# Autodesk Inventor assembly: Arm
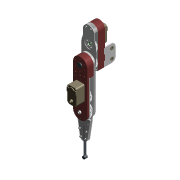
[picture p0: Inventor's stored thumbnail of the model, 180x180]
Saved by Autodesk Inventor 2013 (Build 170138000, 138)
## iProperties
Created: 2013-02-07
Part Number: Arm
Document SubType Name: Assembly
Designer: JohnHenry
Mass: 271.096 g
Surface Area: 817.136 cm^2
Volume: 121.712 cm^3
Density: 2.22735 g/cm^3
Author: JohnHenry
## Documents named in this file (23)
- C:\Users\victor\Desktop\Documents\Inventor\walkPivot\Arm.iam
- C:\Users\victor\Desktop\Documents\Inventor\walkPivot\JointC3_2nd.ipt
- C:\Users\victor\Desktop\Documents\Inventor\walkPivot\JointC3'_2nd.ipt
- C:\Users\victor\Desktop\Documents\Inventor\walkPivot\ベアリング(仮).ipt
- C:\Users\victor\Desktop\Documents\Inventor\walkPivot\RS30x_BottomShaft.ipt
- C:\Users\victor\Desktop\Documents\Inventor\walkPivot\RS30x_ServoHorn.ipt
- C:\Users\victor\Desktop\Documents\Inventor\walkPivot\S75B 40B+0306\デザイン アクセラレータ\平歯車11.ipt
- C:\Users\victor\Desktop\Documents\Inventor\walkPivot\JointC3'cover_2nd.ipt
- C:\Users\victor\Desktop\Documents\Inventor\walkPivot\JointC2_2nd.ipt
- C:\Users\victor\Desktop\Documents\Inventor\walkPivot\S75B 40B+0306\デザイン アクセラレータ\平歯車11_.ipt
- C:\Users\victor\Desktop\Documents\Inventor\walkPivot\JointC3'B_2nd.ipt
- C:\Users\victor\Desktop\Documents\Inventor\walkPivot\JointD0_2nd.ipt
- C:\Users\victor\Desktop\Documents\Inventor\walkPivot\S75B 40B+0306\デザイン アクセラレータ\平歯車11__.ipt
- C:\Users\victor\Desktop\Documents\Inventor\walkPivot\JointD2_2nd.ipt
- C:\Users\victor\Desktop\Documents\Inventor\walkPivot\JointC2cover_2nd.ipt
- C:\Users\victor\Desktop\Documents\Inventor\walkPivot\M2_5mm.ipt
- C:\Users\victor\Desktop\Documents\Inventor\walkPivot\M3_10.ipt
- C:\Users\victor\Desktop\Documents\Inventor\walkPivot\80F-0605.ipt
- C:\Users\victor\Desktop\Documents\Inventor\walkPivot\M1.6_5mm.ipt
- C:\Users\victor\Desktop\Documents\Inventor\walkPivot\shaft6-47.8.ipt
- C:\Users\victor\Desktop\Documents\Inventor\walkPivot\shaft6-19.ipt
- C:\Users\victor\Desktop\Documents\Inventor\walkPivot\JointD0cover_2nd.ipt
- C:\Users\victor\Desktop\Documents\Inventor\walkPivot\JointC3'cover2_2nd.ipt
## Components (81 placed, 20 different names)
1. JointC3_2nd:1 — 挿入:1, 挿入:2, 挿入:3, 挿入:4, 挿入:5, 挿入:6, 挿入:70, 挿入:71, 挿入:72, 挿入:73
2. JointC3'_2nd:1 — 挿入:5, 挿入:6, メイト:2, 角度:1, 挿入:9, 挿入:10, メイト:3, メイト:6, フラッシュ:3, 角度:5, 挿入:60
3. ベアリング(仮):1 — 挿入:3
4. ベアリング(仮):2 — 挿入:2
5. ベアリング(仮):3 — 挿入:4
6. ベアリング(仮):4 — 挿入:1
7. RS30x_BottomShaft:1 — メイト:2, メイト:6, フラッシュ:3, 挿入:13
8. RS30x_ServoHorn:1 — 角度:1, 角度:2, 挿入:8, 挿入:13
9. 平歯車1:1 — 角度:2, 挿入:8, フラッシュ:2, 挿入:66, 挿入:67, 挿入:68, 挿入:69
10. JointC3'cover_2nd:1 — 挿入:9, 挿入:10, 挿入:38, 挿入:39, 挿入:40, 挿入:41, 挿入:53, 挿入:54, 挿入:61, 挿入:86, 挿入:87, 挿入:90, 挿入:91
11. JointC2_2nd:1 — 挿入:11, 挿入:12, メイト:4, メイト:5, フラッシュ:4, 挿入:16, 挿入:17, メイト:7, 角度:5, 角度:6, 挿入:24, 挿入:25, 挿入:74, 挿入:96
12. 平歯車1:2 — メイト:3, フラッシュ:2, 挿入:11, 挿入:12, 挿入:44, 挿入:45, 挿入:46, 挿入:47, 挿入:48, 挿入:49
13. RS30x_BottomShaft:2 — メイト:4, メイト:5, フラッシュ:4, 挿入:14
14. RS30x_ServoHorn:2 — 挿入:14, 角度:4, 挿入:20
15. 平歯車1:3 — 角度:4, フラッシュ:5, 挿入:20, 挿入:62, 挿入:63, 挿入:64, 挿入:65
16. JointC3'B_2nd:1 — 挿入:16, 挿入:17, 挿入:55, 挿入:56, 挿入:57
17. JointD0_2nd:1 — 挿入:18, 挿入:19, フラッシュ:6, メイト:8, メイト:9, 挿入:23, 挿入:26, 挿入:27, 挿入:28, 挿入:29, 挿入:76, 挿入:77, 挿入:78, 挿入:79, 挿入:92
18. 平歯車1:4 — メイト:7, フラッシュ:5, 挿入:18, 挿入:19, 挿入:95
19. JointD2_2nd:1 — フラッシュ:6, メイト:8, メイト:9, 角度:6
20. JointC2cover_2nd:1 — 挿入:24, 挿入:25, 挿入:30, 挿入:31, 挿入:32, 挿入:33, 挿入:34, 挿入:50, 挿入:51, 挿入:52, 挿入:88, 挿入:89
21. M2_5mm:1 — 挿入:31
22. M2_5mm:2 — 挿入:28
23. M2_5mm:3 — 挿入:29
24. M2_5mm:4 — 挿入:32
25. M2_5mm:5 — 挿入:41
26. M2_5mm:6 — 挿入:40
27. M2_5mm:7 — 挿入:33
28. M2_5mm:8 — 挿入:52
29. M2_5mm:9 — 挿入:34
30. M2_5mm:10 — 挿入:30
31. M2_5mm:11 — 挿入:26
32. M2_5mm:12 — 挿入:27
33. M2_5mm:13 — 挿入:50
34. M2_5mm:15 — 挿入:38
35. M2_5mm:16 — 挿入:23
36. M2_5mm:17 — 挿入:39
37. M2_5mm:18 — 挿入:51
38. M2_5mm:20 — 挿入:49
39. M2_5mm:21 — 挿入:48
40. M2_5mm:25 — 挿入:45
41. M2_5mm:26 — 挿入:44
42. M2_5mm:27 — 挿入:47
43. M2_5mm:28 — 挿入:46
44. M2_5mm:29 — 挿入:54
45. M2_5mm:30 — 挿入:53
46. M3_10:1 — 挿入:55
47. M3_10:2 — 挿入:56
48. M3_10:3 — 挿入:57
49. 80F-0605:1 — 挿入:95
50. 80F-0605:3 — 挿入:61
51. 80F-0605:4 — 挿入:60
52. M1.6_5mm:1 — 挿入:62
53. M1.6_5mm:2 — 挿入:64
54. M1.6_5mm:3 — 挿入:65
55. M1.6_5mm:4 — 挿入:63
56. M1.6_5mm:5 — 挿入:67
57. M1.6_5mm:6 — 挿入:66
58. M1.6_5mm:7 — 挿入:68
59. M1.6_5mm:8 — 挿入:69
60. M3_10:4 — 挿入:71
61. M3_10:5 — 挿入:70
62. M3_10:6 — 挿入:73
63. M3_10:7 — 挿入:72
64. shaft6-47.8:1 — 挿入:74
65. shaft6-19:1 — 挿入:96, 挿入:97, 挿入:98
66. JointD0cover_2nd:1 — 挿入:78, 挿入:79, 挿入:81, 挿入:82, 挿入:84, 挿入:85
67. JointD0cover_2nd:2 — 挿入:76, 挿入:77
68. M2_5mm:31 — 挿入:85
69. M2_5mm:32 — 挿入:84
70. M2_5mm:35 — 挿入:81
71. M2_5mm:36 — 挿入:82
72. JointC3'cover2_2nd:1 — 挿入:86, 挿入:87, 挿入:93, 挿入:94
73. M2_5mm:37 — 挿入:89
74. M2_5mm:38 — 挿入:88
75. M2_5mm:39 — 挿入:90
76. M2_5mm:40 — 挿入:91
77. M2_5mm:41 — 挿入:92
78. M2_5mm:42 — 挿入:94
79. M2_5mm:43 — 挿入:93
80. M3_10:8 — 挿入:97
81. M3_10:9 — 挿入:98
## Relationships (102: Insert 84, Mate 8, Angle 5, Flush 5)
- 挿入:1 [Insert]: JointC3_2nd:1 ↔ ベアリング(仮):4
- 挿入:2 [Insert]: JointC3_2nd:1 ↔ ベアリング(仮):2
- 挿入:3 [Insert]: JointC3_2nd:1 ↔ ベアリング(仮):1
- 挿入:4 [Insert]: JointC3_2nd:1 ↔ ベアリング(仮):3
- 挿入:5 [Insert]: JointC3_2nd:1 ↔ JointC3'_2nd:1
- 挿入:6 [Insert]: JointC3_2nd:1 ↔ JointC3'_2nd:1
- メイト:2 [Mate] (0.05 mm): JointC3'_2nd:1 ↔ RS30x_BottomShaft:1
- 角度:1 [Angle] (0 deg): JointC3'_2nd:1 ↔ RS30x_ServoHorn:1
- 角度:2 [Angle] (0 deg): RS30x_ServoHorn:1 ↔ 平歯車1:1
- 挿入:8 [Insert]: RS30x_ServoHorn:1 ↔ 平歯車1:1
- 挿入:9 [Insert]: JointC3'_2nd:1 ↔ JointC3'cover_2nd:1
- 挿入:10 [Insert]: JointC3'_2nd:1 ↔ JointC3'cover_2nd:1
- メイト:3 [Mate]: JointC3'_2nd:1 ↔ 平歯車1:2
- フラッシュ:2 [Flush]: 平歯車1:1 ↔ 平歯車1:2
- 挿入:11 [Insert]: JointC2_2nd:1 ↔ 平歯車1:2
- 挿入:12 [Insert]: JointC2_2nd:1 ↔ 平歯車1:2
- メイト:4 [Mate] (0.05 mm): JointC2_2nd:1 ↔ RS30x_BottomShaft:2
- メイト:5 [Mate] (0.05 mm): JointC2_2nd:1 ↔ RS30x_BottomShaft:2
- メイト:6 [Mate] (0.05 mm): JointC3'_2nd:1 ↔ RS30x_BottomShaft:1
- フラッシュ:3 [Flush]: JointC3'_2nd:1 ↔ RS30x_BottomShaft:1
- 挿入:13 [Insert]: RS30x_BottomShaft:1 ↔ RS30x_ServoHorn:1
- フラッシュ:4 [Flush]: JointC2_2nd:1 ↔ RS30x_BottomShaft:2
- 挿入:14 [Insert]: RS30x_BottomShaft:2 ↔ RS30x_ServoHorn:2
- 角度:4 [Angle] (0 deg): RS30x_ServoHorn:2 ↔ 平歯車1:3
- 挿入:16 [Insert]: JointC2_2nd:1 ↔ JointC3'B_2nd:1
- 挿入:17 [Insert]: JointC2_2nd:1 ↔ JointC3'B_2nd:1
- メイト:7 [Mate]: JointC2_2nd:1 ↔ 平歯車1:4
- フラッシュ:5 [Flush]: 平歯車1:3 ↔ 平歯車1:4
- 挿入:18 [Insert]: JointD0_2nd:1 ↔ 平歯車1:4
- 挿入:19 [Insert]: JointD0_2nd:1 ↔ 平歯車1:4
- 角度:5 [Angle] (0 deg): JointC3'_2nd:1 ↔ JointC2_2nd:1
- フラッシュ:6 [Flush]: JointD0_2nd:1 ↔ JointD2_2nd:1
- メイト:8 [Mate] (0.5 mm): JointD0_2nd:1 ↔ JointD2_2nd:1
- メイト:9 [Mate]: JointD0_2nd:1 ↔ JointD2_2nd:1
- 角度:6 [Angle] (0 deg): JointC2_2nd:1 ↔ JointD2_2nd:1
- 挿入:20 [Insert]: RS30x_ServoHorn:2 ↔ 平歯車1:3
- 挿入:23 [Insert]: JointD0_2nd:1 ↔ M2_5mm:16
- 挿入:24 [Insert]: JointC2_2nd:1 ↔ JointC2cover_2nd:1
- 挿入:25 [Insert]: JointC2_2nd:1 ↔ JointC2cover_2nd:1
- 挿入:26 [Insert]: JointD0_2nd:1 ↔ M2_5mm:11
- 挿入:27 [Insert]: JointD0_2nd:1 ↔ M2_5mm:12
- 挿入:28 [Insert]: JointD0_2nd:1 ↔ M2_5mm:2
- 挿入:29 [Insert]: JointD0_2nd:1 ↔ M2_5mm:3
- 挿入:30 [Insert]: JointC2cover_2nd:1 ↔ M2_5mm:10
- 挿入:31 [Insert]: JointC2cover_2nd:1 ↔ M2_5mm:1
- 挿入:32 [Insert]: JointC2cover_2nd:1 ↔ M2_5mm:4
- 挿入:33 [Insert]: JointC2cover_2nd:1 ↔ M2_5mm:7
- 挿入:34 [Insert]: JointC2cover_2nd:1 ↔ M2_5mm:9
- 挿入:38 [Insert]: JointC3'cover_2nd:1 ↔ M2_5mm:15
- 挿入:39 [Insert]: JointC3'cover_2nd:1 ↔ M2_5mm:17
- 挿入:40 [Insert]: JointC3'cover_2nd:1 ↔ M2_5mm:6
- 挿入:41 [Insert]: JointC3'cover_2nd:1 ↔ M2_5mm:5
- 挿入:44 [Insert]: 平歯車1:2 ↔ M2_5mm:26
- 挿入:45 [Insert]: 平歯車1:2 ↔ M2_5mm:25
- 挿入:46 [Insert]: 平歯車1:2 ↔ M2_5mm:28
- 挿入:47 [Insert]: 平歯車1:2 ↔ M2_5mm:27
- 挿入:48 [Insert]: 平歯車1:2 ↔ M2_5mm:21
- 挿入:49 [Insert]: 平歯車1:2 ↔ M2_5mm:20
- 挿入:50 [Insert]: JointC2cover_2nd:1 ↔ M2_5mm:13
- 挿入:51 [Insert]: JointC2cover_2nd:1 ↔ M2_5mm:18
- 挿入:52 [Insert]: JointC2cover_2nd:1 ↔ M2_5mm:8
- 挿入:53 [Insert]: JointC3'cover_2nd:1 ↔ M2_5mm:30
- 挿入:54 [Insert]: JointC3'cover_2nd:1 ↔ M2_5mm:29
- 挿入:55 [Insert]: JointC3'B_2nd:1 ↔ M3_10:1
- 挿入:56 [Insert]: JointC3'B_2nd:1 ↔ M3_10:2
- 挿入:57 [Insert]: JointC3'B_2nd:1 ↔ M3_10:3
- 挿入:60 [Insert]: JointC3'_2nd:1 ↔ 80F-0605:4
- 挿入:61 [Insert]: JointC3'cover_2nd:1 ↔ 80F-0605:3
- 挿入:62 [Insert]: 平歯車1:3 ↔ M1.6_5mm:1
- 挿入:63 [Insert]: 平歯車1:3 ↔ M1.6_5mm:4
- 挿入:64 [Insert]: 平歯車1:3 ↔ M1.6_5mm:2
- 挿入:65 [Insert]: 平歯車1:3 ↔ M1.6_5mm:3
- 挿入:66 [Insert]: 平歯車1:1 ↔ M1.6_5mm:6
- 挿入:67 [Insert]: 平歯車1:1 ↔ M1.6_5mm:5
- 挿入:68 [Insert]: 平歯車1:1 ↔ M1.6_5mm:7
- 挿入:69 [Insert]: 平歯車1:1 ↔ M1.6_5mm:8
- 挿入:70 [Insert]: JointC3_2nd:1 ↔ M3_10:5
- 挿入:71 [Insert]: JointC3_2nd:1 ↔ M3_10:4
- 挿入:72 [Insert]: JointC3_2nd:1 ↔ M3_10:7
- 挿入:73 [Insert]: JointC3_2nd:1 ↔ M3_10:6
- 挿入:74 [Insert]: JointC2_2nd:1 ↔ shaft6-47.8:1
- 挿入:76 [Insert]: JointD0_2nd:1 ↔ JointD0cover_2nd:2
- 挿入:77 [Insert]: JointD0_2nd:1 ↔ JointD0cover_2nd:2
- 挿入:78 [Insert]: JointD0_2nd:1 ↔ JointD0cover_2nd:1
- 挿入:79 [Insert]: JointD0_2nd:1 ↔ JointD0cover_2nd:1
- 挿入:81 [Insert]: JointD0cover_2nd:1 ↔ M2_5mm:35
- 挿入:82 [Insert]: JointD0cover_2nd:1 ↔ M2_5mm:36
- 挿入:84 [Insert]: JointD0cover_2nd:1 ↔ M2_5mm:32
- 挿入:85 [Insert]: JointD0cover_2nd:1 ↔ M2_5mm:31
- 挿入:86 [Insert]: JointC3'cover_2nd:1 ↔ JointC3'cover2_2nd:1
- 挿入:87 [Insert]: JointC3'cover_2nd:1 ↔ JointC3'cover2_2nd:1
- 挿入:88 [Insert]: JointC2cover_2nd:1 ↔ M2_5mm:38
- 挿入:89 [Insert]: JointC2cover_2nd:1 ↔ M2_5mm:37
- 挿入:90 [Insert]: JointC3'cover_2nd:1 ↔ M2_5mm:39
- 挿入:91 [Insert]: JointC3'cover_2nd:1 ↔ M2_5mm:40
- 挿入:92 [Insert]: JointD0_2nd:1 ↔ M2_5mm:41
- 挿入:93 [Insert]: JointC3'cover2_2nd:1 ↔ M2_5mm:43
- 挿入:94 [Insert]: JointC3'cover2_2nd:1 ↔ M2_5mm:42
- 挿入:95 [Insert]: 平歯車1:4 ↔ 80F-0605:1
- 挿入:96 [Insert]: JointC2_2nd:1 ↔ shaft6-19:1
- 挿入:97 [Insert]: shaft6-19:1 ↔ M3_10:8
- 挿入:98 [Insert]: shaft6-19:1 ↔ M3_10:9
